# Autodesk Inventor assembly: 6P Sprocket
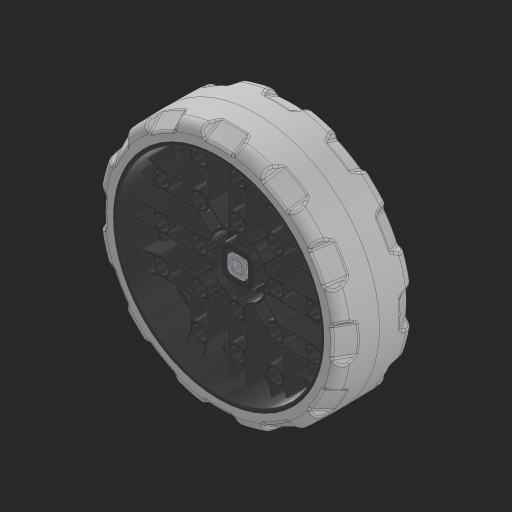
[picture p0: Inventor's stored thumbnail of the model, 512x512]
Saved by Autodesk Inventor 2023 (Build 270158000, 158)
## iProperties
Created: 2022-08-02
Part Number: 6P Sprocket
Document SubType Name: Assembly
Designer: ylu12
Author: ylu12
## Documents named in this file (4)
- C:\Users\ylu12\Documents\GitHub\VEX-CAD-Inventor\Motion\Wheels\Traction Wheel\3.25 Traction AS, Square.iam
- C:\Users\ylu12\Documents\GitHub\VEX-CAD-Inventor\Motion\Wheels\Reference Files\3.25 Traction Antistatic.ipt
- C:\Users\ylu12\Documents\GitHub\VEX-CAD-Inventor\Motion\HS Shaft Adapter Square.ipt
- C:\Users\ylu12\Documents\GitHub\VEX-CAD-Inventor\Motion\Wheels\Traction Wheel.iam
## Components (2 placed, 2 different names)
1. 3.25 Traction Antistatic:1 — Mate:20, Mate:22, Mate:24
2. Square — Mate:30, Mate:31, Flush:9
## Relationships (6: Mate 5, Flush 1)
- Mate:20: 3.25 Traction Antistatic:1
- Mate:22: 3.25 Traction Antistatic:1
- Mate:24: 3.25 Traction Antistatic:1
- Mate:30: Square
- Mate:31: Square
- Flush:9 (-6.35 mm): Square
## Named parameters: Thickness = 8.255 mm
